# Autodesk Inventor assembly: 三組合窗
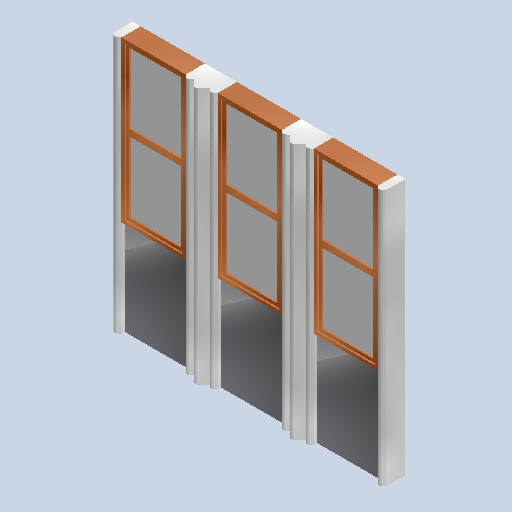
[picture p0: Inventor's stored thumbnail of the model, 512x512]
Saved by Autodesk Inventor 2024.2 (Build 282272000, 272)
## iProperties
Created: 2024-06-02
Part Number: 三組合窗
Document SubType Name: Assembly
Designer: User
Author: User
## Documents named in this file (4)
- C:\Users\User\OneDrive - 國立中山大學\桌面\創客基礎\final_project\三組合窗.iam
- C:\Users\User\OneDrive - 國立中山大學\桌面\創客基礎\final_project\窗.ipt
- C:\Users\User\OneDrive - 國立中山大學\桌面\創客基礎\final_project\窗側柱.ipt
- C:\Users\User\OneDrive - 國立中山大學\桌面\創客基礎\final_project\窗間柱.ipt
## Components (7 placed, 3 different names)
1. 窗:1 — 貼合:2, 貼合:6, 齊平:1, 齊平:2, 齊平:11, 齊平:12
2. 窗:2 — 貼合:1, 貼合:4, 齊平:3, 齊平:4, 齊平:9, 齊平:10
3. 窗:3 — 貼合:3, 貼合:5, 齊平:5, 齊平:6, 齊平:7, 齊平:8
4. 窗側柱:1 — 貼合:6, 齊平:1, 齊平:12
5. 窗側柱:2 — 貼合:5, 齊平:6, 齊平:7
6. 窗間柱:1 — 貼合:3, 貼合:4, 齊平:4, 齊平:5, 齊平:8, 齊平:9
7. 窗間柱:2 — 貼合:1, 貼合:2, 齊平:2, 齊平:3, 齊平:10, 齊平:11
## Relationships (18: Flush 12, Mate 6)
- 貼合:1 [Mate]: 窗:2 ↔ 窗間柱:2
- 貼合:2 [Mate]: 窗:1 ↔ 窗間柱:2
- 貼合:3 [Mate]: 窗:3 ↔ 窗間柱:1
- 貼合:4 [Mate]: 窗:2 ↔ 窗間柱:1
- 貼合:5 [Mate]: 窗:3 ↔ 窗側柱:2
- 貼合:6 [Mate]: 窗:1 ↔ 窗側柱:1
- 齊平:1 [Flush]: 窗:1 ↔ 窗側柱:1
- 齊平:2 [Flush]: 窗:1 ↔ 窗間柱:2
- 齊平:3 [Flush]: 窗:2 ↔ 窗間柱:2
- 齊平:4 [Flush]: 窗:2 ↔ 窗間柱:1
- 齊平:5 [Flush]: 窗:3 ↔ 窗間柱:1
- 齊平:6 [Flush]: 窗:3 ↔ 窗側柱:2
- 齊平:7 [Flush]: 窗:3 ↔ 窗側柱:2
- 齊平:8 [Flush]: 窗:3 ↔ 窗間柱:1
- 齊平:9 [Flush]: 窗:2 ↔ 窗間柱:1
- 齊平:10 [Flush]: 窗:2 ↔ 窗間柱:2
- 齊平:11 [Flush]: 窗:1 ↔ 窗間柱:2
- 齊平:12 [Flush]: 窗:1 ↔ 窗側柱:1
